# Autodesk Inventor assembly: Aschse
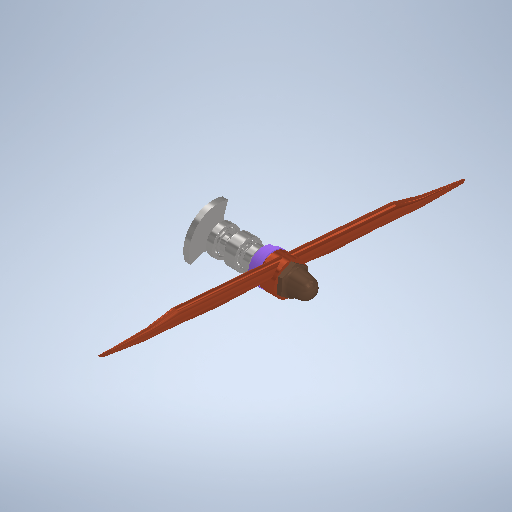
[picture p0: Inventor's stored thumbnail of the model, 512x512]
Saved by Autodesk Inventor 2025 (Build 290162010, 162A)
## iProperties
Created: 2024-07-16
Part Number: Aschse
Document SubType Name: Assembly
Designer: ffogue
Author: ffogue
## Documents named in this file (10)
- C:\Users\ffogue\OneDrive - MuM - OM\Dokumente\Inventor\Boxermotor\Aschse.iam
- C:\Users\ffogue\OneDrive - MuM - OM\Dokumente\Inventor\Boxermotor\Mitnehmer.ipt
- C:\Users\ffogue\OneDrive - MuM - OM\Dokumente\Inventor\Boxermotor\Propeller.ipt
- C:\Users\ffogue\OneDrive - MuM - OM\Dokumente\Inventor\Boxermotor\Spinner.ipt
- C:\Users\ffogue\OneDrive - MuM - OM\Dokumente\Inventor\Content Center Files\R2025\en-US\DIN 625 - T1\DIN 625 T1 - 16003 - 17 x 35 x 8.ipt
- C:\Users\ffogue\OneDrive - MuM - OM\Dokumente\Inventor\Content Center Files\R2025\en-US\DIN 625 - T1\DIN 625 T1 - 6001 - 12 x 28 x 8.ipt
- C:\Users\ffogue\OneDrive - MuM - OM\Dokumente\Inventor\Content Center Files\R2025\en-US\DIN 625 - T3\DIN 625 T3 - 4202 - 15 x 35 x 14.ipt
- C:\Users\ffogue\OneDrive - MuM - OM\Dokumente\Inventor\Boxermotor\Welle.ipt
- C:\Users\ffogue\OneDrive - MuM - OM\Dokumente\Inventor\Boxermotor\Deckscheibe.ipt
- C:\Users\ffogue\OneDrive - MuM - OM\Dokumente\Inventor\Content Center Files\R2025\en-US\DIN 6799\DIN 6799 - 9 10.ipt
## Components (9 placed, 9 different names)
1. Mitnehmer:1 — Mate:1, Insert:1, Mate:6, Insert:5
2. Propeller:1 — Mate:1, Insert:1, Mate:2, Insert:2
3. Spinner:1 — Mate:2, Insert:2
4. DIN 625 - T1 16003 - 17 x 35 x 8:1 — Mate:3, Insert:3
5. DIN 625 - T1 6001 - 12 x 28 x 8:1 — Mate:5, Insert:6
6. DIN 625 - T3 4202 - 15 x 35 x 14:1 — Mate:4, Insert:4
7. Welle:1 — Mate:3, Insert:3, Mate:4, Insert:4, Mate:5, Mate:6, Insert:5, Insert:6, Insert:7, Angle:1, Mate:10
8. Deckscheibe:1
9. DIN 6799 9:1 — Insert:7
## Relationships (15: Mate 7, Insert 7, Angle 1)
- Mate:1: Mitnehmer:1 ↔ Propeller:1
- Insert:1: Mitnehmer:1 ↔ Propeller:1
- Mate:2: Propeller:1 ↔ Spinner:1
- Insert:2: Propeller:1 ↔ Spinner:1
- Mate:3: DIN 625 - T1 16003 - 17 x 35 x 8:1 ↔ Welle:1
- Insert:3: DIN 625 - T1 16003 - 17 x 35 x 8:1 ↔ Welle:1
- Mate:4: DIN 625 - T3 4202 - 15 x 35 x 14:1 ↔ Welle:1
- Insert:4: DIN 625 - T3 4202 - 15 x 35 x 14:1 ↔ Welle:1
- Mate:5: DIN 625 - T1 6001 - 12 x 28 x 8:1 ↔ Welle:1
- Mate:6: Mitnehmer:1 ↔ Welle:1
- Insert:5 (-53 mm): Mitnehmer:1 ↔ Welle:1
- Insert:6: DIN 625 - T1 6001 - 12 x 28 x 8:1 ↔ Welle:1
- Insert:7: Welle:1 ↔ DIN 6799 9:1
- Angle:1 (-135 deg): Welle:1
- Mate:10: Welle:1
